# Autodesk Inventor assembly: Q5_Fan_Assem
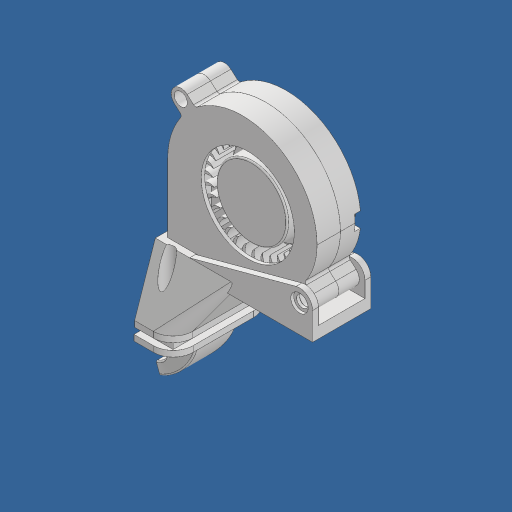
[picture p0: Inventor's stored thumbnail of the model, 512x512]
Saved by Autodesk Inventor 2024.2 (Build 282272000, 272)
## iProperties
Created: 2024-06-06
Part Number: Q5_Fan_Assem
Document SubType Name: Assembly
Designer: Charlie Kendall
Author: Charlie Kendall
## Documents named in this file (4)
- E:\1char\Documents\Q5\Q5_Fan_Assem.iam
- E:\1char\Documents\Q5\Fan_Duct_1.ipt
- E:\1char\Documents\Q5\Fan 5015\Fan 5015.ipt
- E:\1char\Documents\Q5\Fan_Duct_2A.ipt
## Components (3 placed, 3 different names)
1. Fan_Duct_1:1 — Mate:2, Mate:3, Mate:4, Mate:5, Mate:6, Flush:1
2. Fan 5015:1 — Mate:2, Mate:3, Mate:4, Mate:5
3. Fan_Duct_2A:1 — Mate:6, Flush:1
## Relationships (6: Mate 5, Flush 1)
- Mate:2: Fan_Duct_1:1 ↔ Fan 5015:1
- Mate:3: Fan_Duct_1:1 ↔ Fan 5015:1
- Mate:4: Fan_Duct_1:1 ↔ Fan 5015:1
- Mate:5: Fan_Duct_1:1 ↔ Fan 5015:1
- Mate:6: Fan_Duct_1:1 ↔ Fan_Duct_2A:1
- Flush:1: Fan_Duct_1:1 ↔ Fan_Duct_2A:1
